# Autodesk Inventor assembly: saucerAssembly
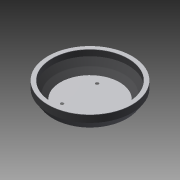
[picture p0: Inventor's stored thumbnail of the model, 180x180]
Saved by Autodesk Inventor 2015 SP1 (Build 190203100, 203)
## iProperties
Created: 2015-02-12
Part Number: saucerAssembly
Document SubType Name: Assembly
Designer: Jostein
Author: Jostein
## Documents named in this file (4)
- C:\Users\Jostein\Desktop\Saucer\saucerAssembly.iam
- C:\Users\Jostein\Desktop\Saucer\bottomPlate.ipt
- C:\Users\Jostein\Desktop\Saucer\foam.ipt
- C:\Users\Jostein\Desktop\Saucer\topRing.ipt
## Components (3 placed, 3 different names)
1. bottomPlate:1
2. foam:1 — Flush:1, Flush:2, Flush:3
3. topRing:1 — Flush:2, Flush:3
## Relationships (3: Flush 3)
- Flush:1: foam:1
- Flush:2: foam:1 ↔ topRing:1
- Flush:3: foam:1 ↔ topRing:1
